# Autodesk Inventor assembly: cellSTORM_v5_baseonly
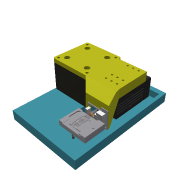
[picture p0: Inventor's stored thumbnail of the model, 180x180]
Saved by Autodesk Inventor 2019.4 (Build 234330000, 330)
## iProperties
Created: 2020-04-25
Part Number: cellSTORM_v5_baseonly
Document SubType Name: Assembly
Designer: diederichbenedict
Author: diederichbenedict
## Documents named in this file (16)
- C:\Users\diederichbenedict\Dropbox\Dokumente\Promotion\PROJECTS\STORMoChip\GITHUB\CAD\Nanoscopy-on-the-cheap\Workspace\cellSTORM_v5_baseonly.iam
- C:\Users\diederichbenedict\Dropbox\Dokumente\Promotion\PROJECTS\STORMoChip\GITHUB\CAD\Nanoscopy-on-the-cheap\Workspace\00_LASER_640nm.ipt
- C:\Users\diederichbenedict\Dropbox\Dokumente\Promotion\PROJECTS\STORMoChip\GITHUB\CAD\Nanoscopy-on-the-cheap\Workspace\00_XY_stage-CHUO_SEIKI_LD-647-R1.iam
- C:\Users\diederichbenedict\Dropbox\Dokumente\Promotion\PROJECTS\STORMoChip\GITHUB\CAD\Nanoscopy-on-the-cheap\Workspace\cellSTORM_laserbeam.ipt
- C:\Users\diederichbenedict\Dropbox\Dokumente\Promotion\PROJECTS\STORMoChip\GITHUB\CAD\Nanoscopy-on-the-cheap\Workspace\02_Nanoscopy_Chip.ipt
- C:\Users\diederichbenedict\Dropbox\Dokumente\Promotion\PROJECTS\STORMoChip\GITHUB\CAD\Nanoscopy-on-the-cheap\Workspace\cellSTORM_nickelplate.ipt
- C:\Users\diederichbenedict\Dropbox\Dokumente\Promotion\PROJECTS\STORMoChip\GITHUB\CAD\Nanoscopy-on-the-cheap\Workspace\00_Ballmagnets_5mm.ipt
- C:\Users\diederichbenedict\Documents\Inventor\Content Center Files\R2019\en-US\DIN 912\DIN 912 - M3 x 0.5 x 25 x 18.ipt
- C:\Users\diederichbenedict\Dropbox\Dokumente\Promotion\PROJECTS\STORMoChip\GITHUB\CAD\Nanoscopy-on-the-cheap\Workspace\cellSTORM_Base_v0_R1.ipt
- C:\Users\diederichbenedict\Dropbox\Dokumente\Promotion\PROJECTS\STORMoChip\GITHUB\CAD\Nanoscopy-on-the-cheap\Workspace\00_KES400.iam
- C:\Users\diederichbenedict\Dropbox\Dokumente\Promotion\PROJECTS\STORMoChip\GITHUB\CAD\Nanoscopy-on-the-cheap\Workspace\cellSTORM_v5_laserstage.ipt
- C:\Users\diederichbenedict\Dropbox\Dokumente\Promotion\PROJECTS\STORMoChip\GITHUB\CAD\Nanoscopy-on-the-cheap\Workspace\cellSTORM_v5_ELECTRONICS.iam
- C:\Users\diederichbenedict\Dropbox\Dokumente\Promotion\PROJECTS\STORMoChip\GITHUB\CAD\Nanoscopy-on-the-cheap\Workspace\00_chip_01_old.ipt
- C:\Users\diederichbenedict\Dropbox\Dokumente\Promotion\PROJECTS\STORMoChip\GITHUB\CAD\Nanoscopy-on-the-cheap\Workspace\cellSTORM_v5_chiptray_old_0.ipt
- C:\Users\diederichbenedict\Dropbox\Dokumente\Promotion\PROJECTS\STORMoChip\GITHUB\CAD\Nanoscopy-on-the-cheap\Workspace\cellSTORM_v5_chiptry_clamp.ipt
- C:\Users\diederichbenedict\Dropbox\Dokumente\Promotion\PROJECTS\STORMoChip\GITHUB\CAD\Nanoscopy-on-the-cheap\Workspace\00_Laser_532nm_200mw.ipt
## Components (19 placed, 15 different names)
1. 00_LASER_640nm:1 — Insert:2, Angle:6, Mate:7, Mate:6, Flush:1, Angle:7, Flush:27
2. 00_XY_stage-CHUO_SEIKI_LD-647-R1:1 [sub-assembly] — Insert:1, Angle:1, Mate:6, Flush:1, Flush:10, Flush:11
3. cellSTORM_laserbeam:1 — Insert:2, Insert:3, Insert:7, Insert:16, Mate:27
4. 02_Nanoscopy_Chip:1 — Insert:3, Angle:2, Mate:9
5. cellSTORM_nickelplate:1 — Mate:9
6. 00_Ballmagnets_5mm:1
7. DIN 912 - replaced by DIN EN ISO 4762 M3 x 25:1 — Insert:4
8. 00_Ballmagnets_5mm:2
9. DIN 912 - replaced by DIN EN ISO 4762 M3 x 25:2 — Insert:13
10. 00_Ballmagnets_5mm:3
11. DIN 912 - replaced by DIN EN ISO 4762 M3 x 25:3 — Insert:14
12. cellSTORM_Base_v0_R1:1 — Insert:1, Angle:1, Angle:2, Insert:4, Angle:6, Mate:7, Insert:13, Insert:14, Flush:23
13. 00_KES400:1 [sub-assembly] — Insert:7, Angle:7, Mate:27, Mate:28
14. cellSTORM_v5_laserstage:1 — Flush:10, Flush:11
15. cellSTORM_v5_ELECTRONICS:1 [sub-assembly]
16. 00_chip_01_old:1 — Flush:22, Insert:16
17. cellSTORM_v5_chiptray_old_0:1 — Flush:22, Flush:23, Flush:24, Flush:25
18. cellSTORM_v5_chiptry_clamp:1 — Flush:24, Flush:25
19. 00_Laser_532nm_200mw:1 — Mate:28, Flush:27
## Relationships (29: Mate 9, Insert 8, Flush 8, Angle 4)
- [Mate]: 02_Nanoscopy_Chip:1 ↔ cellSTORM_nickelplate:1
- [Mate]: 00_Ballmagnets_5mm:1 ↔ DIN 912 - replaced by DIN EN ISO 4762 M3 x 25:1
- [Mate]: 00_Ballmagnets_5mm:2 ↔ DIN 912 - replaced by DIN EN ISO 4762 M3 x 25:2
- [Mate]: 00_Ballmagnets_5mm:3 ↔ DIN 912 - replaced by DIN EN ISO 4762 M3 x 25:3
- Insert:1: 00_XY_stage-CHUO_SEIKI_LD-647-R1:1 ↔ cellSTORM_Base_v0_R1:1
- Angle:1 (90 deg): 00_XY_stage-CHUO_SEIKI_LD-647-R1:1 ↔ cellSTORM_Base_v0_R1:1
- Insert:2 (-10 mm): 00_LASER_640nm:1 ↔ cellSTORM_laserbeam:1
- Insert:3 (5 mm): cellSTORM_laserbeam:1 ↔ 02_Nanoscopy_Chip:1
- Angle:2 (180 deg): 02_Nanoscopy_Chip:1 ↔ cellSTORM_Base_v0_R1:1
- Insert:4 (-15 mm): DIN 912 - replaced by DIN EN ISO 4762 M3 x 25:1 ↔ cellSTORM_Base_v0_R1:1
- Angle:6 (0 deg): 00_LASER_640nm:1 ↔ cellSTORM_Base_v0_R1:1
- Mate:7 (1 mm): 00_LASER_640nm:1 ↔ cellSTORM_Base_v0_R1:1
- Mate:6 (10 mm): 00_LASER_640nm:1 ↔ 00_XY_stage-CHUO_SEIKI_LD-647-R1:1
- Flush:1 (-5 mm): 00_LASER_640nm:1 ↔ 00_XY_stage-CHUO_SEIKI_LD-647-R1:1
- Insert:7: cellSTORM_laserbeam:1 ↔ 00_KES400:1
- Angle:7 (0 deg): 00_LASER_640nm:1 ↔ 00_KES400:1
- Insert:13 (-15 mm): DIN 912 - replaced by DIN EN ISO 4762 M3 x 25:2 ↔ cellSTORM_Base_v0_R1:1
- Insert:14 (-15 mm): DIN 912 - replaced by DIN EN ISO 4762 M3 x 25:3 ↔ cellSTORM_Base_v0_R1:1
- Mate:9: 02_Nanoscopy_Chip:1 ↔ cellSTORM_nickelplate:1
- Flush:10: 00_XY_stage-CHUO_SEIKI_LD-647-R1:1 ↔ cellSTORM_v5_laserstage:1
- Flush:11: 00_XY_stage-CHUO_SEIKI_LD-647-R1:1 ↔ cellSTORM_v5_laserstage:1
- Flush:22: 00_chip_01_old:1 ↔ cellSTORM_v5_chiptray_old_0:1
- Flush:23 (10 mm): cellSTORM_Base_v0_R1:1 ↔ cellSTORM_v5_chiptray_old_0:1
- Insert:16: cellSTORM_laserbeam:1 ↔ 00_chip_01_old:1
- Flush:24: cellSTORM_v5_chiptray_old_0:1 ↔ cellSTORM_v5_chiptry_clamp:1
- Flush:25: cellSTORM_v5_chiptray_old_0:1 ↔ cellSTORM_v5_chiptry_clamp:1
- Mate:27: cellSTORM_laserbeam:1 ↔ 00_KES400:1
- Mate:28: 00_KES400:1 ↔ 00_Laser_532nm_200mw:1
- Flush:27: 00_LASER_640nm:1 ↔ 00_Laser_532nm_200mw:1
## Named parameters: d2_d162 = 0 mm, d3_d162 = 0 mm
